# Autodesk Inventor assembly: one side of drive_MIR
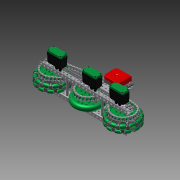
[picture p0: Inventor's stored thumbnail of the model, 180x180]
Saved by Autodesk Inventor 2014 SP1 (Build 180222100, 222)
## iProperties
Created: 2014-03-07
Part Number: one side of drive_MIR
Document SubType Name: Assembly
Designer: Ryan
Author: Ryan
## Documents named in this file (26)
- C:\Users\Ryan\Desktop\sw\toss up 5th A bot\drive\one side of drive_MIR.iam
- C:\Users\Ryan\Desktop\sw\lib\Aperture VEX CAD Library\Metal\C Channel\2 x 25.ipt
- C:\Users\Ryan\Desktop\sw\lib\Aperture VEX CAD Library\Bearing Blocks\Bearing Block with screws.iam
- C:\Users\Ryan\Desktop\sw\toss up 5th A bot\drive\wheel assembly.iam
- C:\Users\Ryan\Desktop\sw\toss up 5th A bot\drive\varsity wheel with sprocket.iam
- C:\Users\Ryan\Desktop\sw\lib\Aperture VEX CAD Library\Standoffs\BEAM-2000.ipt
- C:\Users\Ryan\Desktop\sw\lib\Aperture VEX CAD Library\Metal\C Channel\5 x 5.ipt
- C:\Users\Ryan\Desktop\sw\lib\Super Sonic Sparks VEX CAD Library\Motors & Sensors\Optical Shaft (Quadrature) Encoder.iam
- C:\Users\Ryan\Desktop\sw\lib\Aperture VEX CAD Library\Spacers\SPACER-0500-0125.ipt
- C:\Users\Ryan\Desktop\sw\lib\Aperture VEX CAD Library\Hardware\8-32\8-32_.375.ipt
- C:\Users\Ryan\Desktop\sw\lib\Aperture VEX CAD Library\Hardware\8-32\8-32 nylock.ipt
- C:\Users\Ryan\Desktop\sw\lib\Aperture VEX CAD Library\Hardware\8-32\8-32_1.500.ipt
- C:\Users\Ryan\Desktop\sw\lib\Aperture VEX CAD Library\Spacers\SPACER-0500-0500.ipt
- C:\Users\Ryan\Desktop\sw\lib\Aperture VEX CAD Library\Spacers\SPACER-0500-0375.ipt
- C:\Users\Ryan\Desktop\sw\lib\Aperture VEX CAD Library\Sprockets\green\High Strength 12-Tooth Sprocket.ipt
- C:\Users\Ryan\Desktop\sw\lib\Aperture VEX CAD Library\Bearing Blocks\Bearing Block.ipt
- C:\Users\Ryan\Desktop\sw\lib\Aperture VEX CAD Library\Hardware\8-32\8-32_.500.ipt
- C:\Users\Ryan\Desktop\sw\lib\Aperture VEX CAD Library\Hardware\Shaft Collar.ipt
- C:\Users\Ryan\Desktop\sw\lib\Aperture VEX CAD Library\Bearing Blocks\Pillow Block.ipt
- C:\Users\Ryan\Desktop\sw\lib\Aperture VEX CAD Library\Spacers\thin\SPACER-0320-0125.ipt
- C:\Users\Ryan\Desktop\sw\lib\Super Sonic Sparks VEX CAD Library\Motors & Sensors\2-Wire Motor 393-Without Wire.iam
- C:\Users\Ryan\Desktop\sw\lib\Aperture VEX CAD Library\Hardware\6-32\6-32_.250.ipt
- C:\Users\Ryan\Desktop\sw\lib\Aperture VEX CAD Library\Hardware\8-32\8-32 nylock_MIR13.ipt
- C:\Users\Ryan\Desktop\sw\lib\Aperture VEX CAD Library\Shaft\3.7 in shaft.ipt
- C:\Users\Ryan\Desktop\sw\lib\Aperture VEX CAD Library\Sprockets\HS Sprockets\High strength Chain Link.ipt
- C:\Users\Ryan\Desktop\sw\toss up 5th A bot\drive\one side of drive\Design Accelerator\V-Belt transmission1.iam
## Components (178 placed, 25 different names)
1. 2 x 25:1 — Mate:2, Mate:1, Mate:4, Mate:3, Mate:13, Mate:12, Mate:11, Mate:16, Mate:15, Mate:14, Flush:2, Flush:1, Mate:105, Angle:1, Mate:104, Mate:118, Mate:120, Mate:124, Mate:125
2. wheel assembly:1 [sub-assembly] — Mate:20, Mate:5, Mate:92
3. wheel assembly:2 [sub-assembly] — Mate:78, Mate:18, Mate:7
4. varsity wheel with sprocket:1 [sub-assembly] — Flush:4, Mate:19, Mate:10
5. BEAM-2000:1 — Mate:13, Mate:12, Mate:11, Mate:115, Mate:117
6. BEAM-2000:2 — Mate:16, Mate:15, Mate:14, Mate:17, Mate:119, Mate:121
7. 2 x 25:2 — Flush:2, Flush:1, Mate:17, Flush:5, Mate:102, Flush:3, Mate:79, Mate:77, Mate:80, Mate:86, Mate:84, Mate:88, Mate:91, Mate:90, Mate:89, Mate:95, Mate:93, Mate:97, Mate:101, Mate:108, Mate:107, Mate:106, Mate:111, Mate:110, Mate:109, Mate:113, Mate:116, Mate:122, Mate:129, Mate:128, Mate:127, Mate:133
8. 5 x 5:1 — Flush:5, Mate:102, Flush:3, Mate:24, Mate:23, Mate:22, Mate:27, Mate:26, Mate:31, Mate:36, Mate:34, Mate:41, Mate:47, Mate:45, Mate:49, Angle:2
9. Optical Shaft (Quadrature) Encoder:1 [sub-assembly] — Mate:24, Mate:23, Mate:22, Mate:25, Mate:33, Mate:44, Mate:46, Mate:137, Flush:7, Mate:136
10. 8-32_1.500:1 — Mate:36, Mate:34, Mate:43, Mate:42
11. SPACER-0500-0500:1 — Mate:43, Mate:38, Mate:37, Mate:39
12. SPACER-0500-0500:2 — Mate:38, Mate:37, Mate:40
13. SPACER-0500-0375:1 — Mate:42, Mate:41, Mate:40, Mate:39
14. High Strength 12-Tooth Sprocket:1 — Flush:4, Mate:44, Mate:53, Mate:52, Mate:139
15. Bearing Block:1 — Mate:47, Mate:46, Mate:45, Mate:48, Mate:50, Mate:75
16. Shaft Collar:1 — Mate:53, Mate:52, Mate:55, Mate:54
17. SPACER-0500-0500:3 — Mate:55, Mate:54, Mate:57, Mate:56, Mate:76
18. SPACER-0500-0500:4 — Mate:57, Mate:56, Mate:58, Mate:62, Mate:61
19. Pillow Block:1 — Mate:105, Angle:1, Mate:58, Mate:103, Mate:70, Mate:72, Mate:71
20. SPACER-0320-0125:1 — Mate:62, Mate:61, Mate:64, Mate:63
21. SPACER-0320-0125:2 — Mate:64, Mate:63
22. SPACER-0500-0375:2 — Mate:76, Mate:75
23. Bearing Block:2 — Mate:79, Mate:78, Mate:77, Mate:81, Mate:83, Mate:85
24. 2-Wire Motor 393-Without Wire:1 [sub-assembly] — Mate:86, Mate:85, Mate:84, Mate:87
25. 8-32_.375:3 — Mate:108, Mate:107, Mate:106, Mate:114
26. 8-32_.375:4 — Mate:111, Mate:110, Mate:109, Mate:112
27. 8-32 nylock_MIR13:1 — Mate:113, Mate:112, Flush:6
28. 8-32 nylock:6 — Flush:6, Mate:114
29. 8-32_.375:5 — Mate:116, Mate:115
30. 8-32_.375:6 — Mate:118, Mate:117
31. 8-32_.375:7 — Mate:120, Mate:119
32. 8-32_.375:8 — Mate:122, Mate:121
33. 3.7 in shaft:1 — Mate:137, Flush:7, Mate:136
34. High strength Chain Link:1 — Angle:2, Mate:139
35. V-Belt transmission:1 [sub-assembly]
36. High strength Chain Link:2
37. High strength Chain Link:3
38. High strength Chain Link:4
39. High strength Chain Link:5
40. High strength Chain Link:6
41. High strength Chain Link:7
42. High strength Chain Link:8
43. High strength Chain Link:9
44. High strength Chain Link:10
45. High strength Chain Link:11
46. High strength Chain Link:12
47. High strength Chain Link:13
48. High strength Chain Link:14
49. High strength Chain Link:15
50. High strength Chain Link:16
51. High strength Chain Link:17
52. High strength Chain Link:18
53. High strength Chain Link:19
54. High strength Chain Link:20
55. High strength Chain Link:21
56. High strength Chain Link:22
57. High strength Chain Link:23
58. High strength Chain Link:24
59. High strength Chain Link:25
60. High strength Chain Link:26
61. High strength Chain Link:27
62. High strength Chain Link:28
63. High strength Chain Link:29
64. High strength Chain Link:30
65. High strength Chain Link:31
66. High strength Chain Link:32
67. High strength Chain Link:33
68. High strength Chain Link:34
69. High strength Chain Link:35
70. High strength Chain Link:36
71. High strength Chain Link:37
72. High strength Chain Link:38
73. High strength Chain Link:39
74. High strength Chain Link:40
75. High strength Chain Link:41
76. High strength Chain Link:42
77. High strength Chain Link:43
78. High strength Chain Link:44
79. High strength Chain Link:45
80. High strength Chain Link:46
81. High strength Chain Link:47
82. High strength Chain Link:48
83. High strength Chain Link:49
84. High strength Chain Link:50
85. High strength Chain Link:51
86. High strength Chain Link:52
87. High strength Chain Link:53
88. High strength Chain Link:54
89. High strength Chain Link:55
90. High strength Chain Link:56
91. High strength Chain Link:57
92. High strength Chain Link:58
93. High strength Chain Link:59
94. High strength Chain Link:60
95. High strength Chain Link:61
96. High strength Chain Link:62
97. High strength Chain Link:63
98. High strength Chain Link:64
99. High strength Chain Link:65
100. High strength Chain Link:66
101. High strength Chain Link:67
102. High strength Chain Link:68
103. High strength Chain Link:69
104. High strength Chain Link:70
105. High strength Chain Link:71
106. High strength Chain Link:72
107. High strength Chain Link:73
108. High strength Chain Link:74
109. High strength Chain Link:75
110. High strength Chain Link:76
111. High strength Chain Link:77
112. High strength Chain Link:78
113. High strength Chain Link:79
114. High strength Chain Link:80
115. High strength Chain Link:81
116. High strength Chain Link:82
117. High strength Chain Link:83
118. High strength Chain Link:84
119. High strength Chain Link:85
120. SPACER-0500-0125:1 — Mate:27, Mate:26, Mate:25, Mate:30, Mate:32
121. 8-32_.375:1 — Mate:31, Mate:30
122. 8-32 nylock:1 — Mate:33, Mate:32
123. SPACER-0500-0125:2
124. 8-32_.375:11
125. 8-32 nylock:9
126. 8-32_.500:2 — Mate:81, Mate:80, Mate:82
127. 8-32 nylock:4 — Mate:83, Mate:82
128. 6-32_.250:1 — Mate:88, Mate:87
129. 8-32_.500:4
130. 8-32 nylock:10
131. 6-32_.250:3
132. 8-32_.500:1 — Mate:49, Mate:48, Mate:51
133. 8-32 nylock:2 — Mate:51, Mate:50
134. 8-32_.500:6
135. 8-32 nylock:12
136. 8-32_.375:2 — Mate:72, Mate:71
137. SPACER-0500-0500:6 — Mate:103, Mate:66, Mate:65
138. SPACER-0500-0500:7 — Mate:70, Mate:68, Mate:67, Mate:66, Mate:65
139. SPACER-0500-0500:5 — Mate:68, Mate:67, Mate:74
140. 8-32 nylock:3 — Mate:104, Mate:74
141. 8-32_.375:12
142. SPACER-0500-0500:8
143. SPACER-0500-0500:9
144. SPACER-0500-0500:10
145. 8-32 nylock:13
146. Bearing Block with screws:1 [sub-assembly] — Mate:2, Mate:1, Mate:4, Mate:3, Mate:20, Mate:5, Mate:123, Mate:126
147. 8-32 nylock:8 — Mate:126, Mate:125
148. 8-32 nylock:7 — Mate:124, Mate:123
149. Bearing Block with screws:2 [sub-assembly] — Mate:19, Mate:10
150. 8-32 nylock:14
151. 8-32 nylock:15
152. Bearing Block with screws:3 [sub-assembly] — Mate:18, Mate:7
153. 8-32 nylock:16
154. 8-32 nylock:17
155. 8-32_.375:9 — Mate:129, Mate:128, Mate:127, Mate:132
156. 8-32_.375:10 — Mate:135, Mate:134
157. SPACER-0500-0375:4 — Mate:132, Mate:131, Mate:130, Mate:135, Mate:134
158. SPACER-0500-0375:3 — Mate:133, Mate:131, Mate:130
159. 8-32_.375:13
160. 8-32_.375:14
161. SPACER-0500-0375:5
162. SPACER-0500-0375:6
163. 2-Wire Motor 393-Without Wire:2 [sub-assembly] — Mate:95, Mate:94, Mate:93, Mate:100
164. Bearing Block:3 — Mate:92, Mate:91, Mate:90, Mate:89, Mate:94, Mate:96, Mate:98
165. 2-Wire Motor 393-Without Wire:3 [sub-assembly]
166. Bearing Block:4
167. 6-32_.250:2 — Mate:101, Mate:100
168. 8-32 nylock:5 — Mate:99, Mate:98
169. 8-32_.500:3 — Mate:97, Mate:96, Mate:99
170. 6-32_.250:4
171. 8-32 nylock:11
172. 8-32_.500:5
173. 6-32_.250:5
174. 8-32 nylock:18
175. 8-32_.500:7
176. 6-32_.250:6
177. 8-32 nylock:19
178. 8-32_.500:8
## Component patterns: (2 elements, first: SPACER-0500-0125:1 + 8-32_.375:1 + 8-32 nylock:1), (2 elements, first: 8-32_.500:2 + 8-32 nylock:4 + 6-32_.250:1), (2 elements, first: 8-32_.500:1 + 8-32 nylock:2), (2 elements, first: 8-32_.375:2 + SPACER-0500-0500:6 + SPACER-0500-0500:7 + SPACER-0500-0500:5 + 8-32 nylock:3), (3 elements, first: Bearing Block with screws:1 + 8-32 nylock:8 + 8-32 nylock:7), (2 elements, first: 8-32_.375:9 + 8-32_.375:10 + SPACER-0500-0375:4 + SPACER-0500-0375:3), (2 elements, first: 2-Wire Motor 393-Without Wire:2 + Bearing Block:3), (2 elements, first: 6-32_.250:2 + 8-32 nylock:5 + 8-32_.500:3), Component Pattern 3:2 (2 elements)
## Relationships (136: Mate 126, Flush 8, Angle 2)
- Mate:2 (2.3114 mm): 2 x 25:1 ↔ Bearing Block with screws:1
- Mate:1: 2 x 25:1 ↔ Bearing Block with screws:1
- Mate:4 (2.3114 mm): 2 x 25:1 ↔ Bearing Block with screws:1
- Mate:3 (2.3114 mm): 2 x 25:1 ↔ Bearing Block with screws:1
- Mate:20: wheel assembly:1 ↔ Bearing Block with screws:1
- Mate:5: wheel assembly:1 ↔ Bearing Block with screws:1
- Mate:13 (2.3114 mm): 2 x 25:1 ↔ BEAM-2000:1
- Mate:12 (2.3114 mm): 2 x 25:1 ↔ BEAM-2000:1
- Mate:11: 2 x 25:1 ↔ BEAM-2000:1
- Mate:16 (2.3114 mm): 2 x 25:1 ↔ BEAM-2000:2
- Mate:15 (2.3114 mm): 2 x 25:1 ↔ BEAM-2000:2
- Mate:14: 2 x 25:1 ↔ BEAM-2000:2
- Flush:2: 2 x 25:1 ↔ 2 x 25:2
- Flush:1: 2 x 25:1 ↔ 2 x 25:2
- Mate:17: BEAM-2000:2 ↔ 2 x 25:2
- Flush:5: 2 x 25:2 ↔ 5 x 5:1
- Mate:102: 2 x 25:2 ↔ 5 x 5:1
- Flush:3: 2 x 25:2 ↔ 5 x 5:1
- Mate:24 (-10.3886 mm): 5 x 5:1 ↔ Optical Shaft (Quadrature) Encoder:1
- Mate:23 (3.175 mm): 5 x 5:1 ↔ Optical Shaft (Quadrature) Encoder:1
- Mate:22 (-2.3114 mm): 5 x 5:1 ↔ Optical Shaft (Quadrature) Encoder:1
- Mate:27 (2.3114 mm): 5 x 5:1 ↔ SPACER-0500-0125:1
- Mate:26 (2.3114 mm): 5 x 5:1 ↔ SPACER-0500-0125:1
- Mate:25: Optical Shaft (Quadrature) Encoder:1 ↔ SPACER-0500-0125:1
- Mate:31: 5 x 5:1 ↔ 8-32_.375:1
- Mate:30: SPACER-0500-0125:1 ↔ 8-32_.375:1
- Mate:33: Optical Shaft (Quadrature) Encoder:1 ↔ 8-32 nylock:1
- Mate:32: SPACER-0500-0125:1 ↔ 8-32 nylock:1
- Mate:36 (2.3114 mm): 5 x 5:1 ↔ 8-32_1.500:1
- Mate:34 (2.3114 mm): 5 x 5:1 ↔ 8-32_1.500:1
- Mate:43: 8-32_1.500:1 ↔ SPACER-0500-0500:1
- Mate:38: SPACER-0500-0500:1 ↔ SPACER-0500-0500:2
- Mate:37: SPACER-0500-0500:1 ↔ SPACER-0500-0500:2
- Mate:42: 8-32_1.500:1 ↔ SPACER-0500-0375:1
- Mate:41: 5 x 5:1 ↔ SPACER-0500-0375:1
- Mate:40: SPACER-0500-0500:2 ↔ SPACER-0500-0375:1
- Mate:39: SPACER-0500-0500:1 ↔ SPACER-0500-0375:1
- Flush:4: varsity wheel with sprocket:1 ↔ High Strength 12-Tooth Sprocket:1
- Mate:44: Optical Shaft (Quadrature) Encoder:1 ↔ High Strength 12-Tooth Sprocket:1
- Mate:47 (2.3114 mm): 5 x 5:1 ↔ Bearing Block:1
- Mate:46: Optical Shaft (Quadrature) Encoder:1 ↔ Bearing Block:1
- Mate:45: 5 x 5:1 ↔ Bearing Block:1
- Mate:49: 5 x 5:1 ↔ 8-32_.500:1
- Mate:48: Bearing Block:1 ↔ 8-32_.500:1
- Mate:51: 8-32_.500:1 ↔ 8-32 nylock:2
- Mate:50: Bearing Block:1 ↔ 8-32 nylock:2
- Mate:53: High Strength 12-Tooth Sprocket:1 ↔ Shaft Collar:1
- Mate:52: High Strength 12-Tooth Sprocket:1 ↔ Shaft Collar:1
- Mate:55: Shaft Collar:1 ↔ SPACER-0500-0500:3
- Mate:54: Shaft Collar:1 ↔ SPACER-0500-0500:3
- Mate:57: SPACER-0500-0500:3 ↔ SPACER-0500-0500:4
- Mate:56: SPACER-0500-0500:3 ↔ SPACER-0500-0500:4
- Mate:105 (2.3114 mm): 2 x 25:1 ↔ Pillow Block:1
- Angle:1 (180 deg): 2 x 25:1 ↔ Pillow Block:1
- Mate:58: SPACER-0500-0500:4 ↔ Pillow Block:1
- Mate:62: SPACER-0500-0500:4 ↔ SPACER-0320-0125:1
- Mate:61: SPACER-0500-0500:4 ↔ SPACER-0320-0125:1
- Mate:64: SPACER-0320-0125:1 ↔ SPACER-0320-0125:2
- Mate:63: SPACER-0320-0125:1 ↔ SPACER-0320-0125:2
- Mate:103: Pillow Block:1 ↔ SPACER-0500-0500:6
- Mate:70: Pillow Block:1 ↔ SPACER-0500-0500:7
- Mate:68: SPACER-0500-0500:7 ↔ SPACER-0500-0500:5
- Mate:67: SPACER-0500-0500:7 ↔ SPACER-0500-0500:5
- Mate:66: SPACER-0500-0500:6 ↔ SPACER-0500-0500:7
- Mate:65: SPACER-0500-0500:6 ↔ SPACER-0500-0500:7
- Mate:72: Pillow Block:1 ↔ 8-32_.375:2
- Mate:71: Pillow Block:1 ↔ 8-32_.375:2
- Mate:104: 2 x 25:1 ↔ 8-32 nylock:3
- Mate:74: SPACER-0500-0500:5 ↔ 8-32 nylock:3
- Mate:76: SPACER-0500-0500:3 ↔ SPACER-0500-0375:2
- Mate:75: Bearing Block:1 ↔ SPACER-0500-0375:2
- Mate:79 (2.3114 mm): 2 x 25:2 ↔ Bearing Block:2
- Mate:78: wheel assembly:2 ↔ Bearing Block:2
- Mate:77: 2 x 25:2 ↔ Bearing Block:2
- Mate:81: Bearing Block:2 ↔ 8-32_.500:2
- Mate:80: 2 x 25:2 ↔ 8-32_.500:2
- Mate:83: Bearing Block:2 ↔ 8-32 nylock:4
- Mate:82: 8-32_.500:2 ↔ 8-32 nylock:4
- Mate:86 (2.3114 mm): 2 x 25:2 ↔ 2-Wire Motor 393-Without Wire:1
- Mate:85: Bearing Block:2 ↔ 2-Wire Motor 393-Without Wire:1
- Mate:84: 2 x 25:2 ↔ 2-Wire Motor 393-Without Wire:1
- Mate:88: 2 x 25:2 ↔ 6-32_.250:1
- Mate:87: 2-Wire Motor 393-Without Wire:1 ↔ 6-32_.250:1
- Mate:92: wheel assembly:1 ↔ Bearing Block:3
- Mate:91 (2.3114 mm): 2 x 25:2 ↔ Bearing Block:3
- Mate:90 (2.3114 mm): 2 x 25:2 ↔ Bearing Block:3
- Mate:89: 2 x 25:2 ↔ Bearing Block:3
- Mate:95 (2.3114 mm): 2 x 25:2 ↔ 2-Wire Motor 393-Without Wire:2
- Mate:94: 2-Wire Motor 393-Without Wire:2 ↔ Bearing Block:3
- Mate:93: 2 x 25:2 ↔ 2-Wire Motor 393-Without Wire:2
- Mate:97: 2 x 25:2 ↔ 8-32_.500:3
- Mate:96: Bearing Block:3 ↔ 8-32_.500:3
- Mate:99: 8-32 nylock:5 ↔ 8-32_.500:3
- Mate:98: Bearing Block:3 ↔ 8-32 nylock:5
- Mate:101: 2 x 25:2 ↔ 6-32_.250:2
- Mate:100: 2-Wire Motor 393-Without Wire:2 ↔ 6-32_.250:2
- Mate:108 (2.3114 mm): 2 x 25:2 ↔ 8-32_.375:3
- Mate:107 (2.3114 mm): 2 x 25:2 ↔ 8-32_.375:3
- Mate:106: 2 x 25:2 ↔ 8-32_.375:3
- Mate:111: 2 x 25:2 ↔ 8-32_.375:4
- Mate:110 (2.3114 mm): 2 x 25:2 ↔ 8-32_.375:4
- Mate:109 (2.3114 mm): 2 x 25:2 ↔ 8-32_.375:4
- Mate:113 (2.3368 mm): 2 x 25:2 ↔ 8-32 nylock_MIR13:1
- Mate:112: 8-32_.375:4 ↔ 8-32 nylock_MIR13:1
- Flush:6: 8-32 nylock_MIR13:1 ↔ 8-32 nylock:6
- Mate:114: 8-32_.375:3 ↔ 8-32 nylock:6
- Mate:116: 2 x 25:2 ↔ 8-32_.375:5
- Mate:115: BEAM-2000:1 ↔ 8-32_.375:5
- Mate:118: 2 x 25:1 ↔ 8-32_.375:6
- Mate:117: BEAM-2000:1 ↔ 8-32_.375:6
- Mate:120: 2 x 25:1 ↔ 8-32_.375:7
- Mate:119: BEAM-2000:2 ↔ 8-32_.375:7
- Mate:122: 2 x 25:2 ↔ 8-32_.375:8
- Mate:121: BEAM-2000:2 ↔ 8-32_.375:8
- Mate:124: 2 x 25:1 ↔ 8-32 nylock:7
- Mate:123: Bearing Block with screws:1 ↔ 8-32 nylock:7
- Mate:126: Bearing Block with screws:1 ↔ 8-32 nylock:8
- Mate:125: 2 x 25:1 ↔ 8-32 nylock:8
- Mate:129: 2 x 25:2 ↔ 8-32_.375:9
- Mate:128 (2.3114 mm): 2 x 25:2 ↔ 8-32_.375:9
- Mate:127 (2.3114 mm): 2 x 25:2 ↔ 8-32_.375:9
- Mate:133: 2 x 25:2 ↔ SPACER-0500-0375:3
- Mate:132: 8-32_.375:9 ↔ SPACER-0500-0375:4
- Mate:131: SPACER-0500-0375:4 ↔ SPACER-0500-0375:3
- Mate:130: SPACER-0500-0375:4 ↔ SPACER-0500-0375:3
- Mate:135: 8-32_.375:10 ↔ SPACER-0500-0375:4
- Mate:134: 8-32_.375:10 ↔ SPACER-0500-0375:4
- Mate:137: Optical Shaft (Quadrature) Encoder:1 ↔ 3.7 in shaft:1
- Flush:7: Optical Shaft (Quadrature) Encoder:1 ↔ 3.7 in shaft:1
- Mate:136 [Flush]: Optical Shaft (Quadrature) Encoder:1 ↔ 3.7 in shaft:1
- Angle:2 (133 deg): 5 x 5:1 ↔ High strength Chain Link:1
- Mate:139: High Strength 12-Tooth Sprocket:1 ↔ High strength Chain Link:1
- Mate:18: wheel assembly:2 ↔ Bearing Block with screws:3
- Mate:7: wheel assembly:2 ↔ Bearing Block with screws:3
- Mate:19: varsity wheel with sprocket:1 ↔ Bearing Block with screws:2
- Mate:10: varsity wheel with sprocket:1 ↔ Bearing Block with screws:2
